# Autodesk Inventor assembly: default_motor_asembly
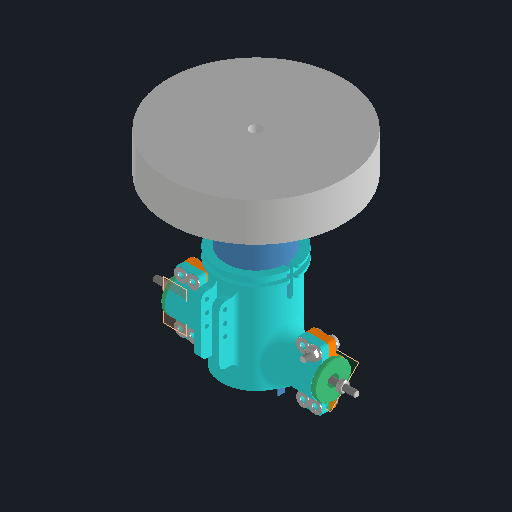
[picture p0: Inventor's stored thumbnail of the model, 512x512]
Saved by Autodesk Inventor 2024 (Build 280153000, 153)
## iProperties
Created: 2023-05-13
Part Number: default_motor_asembly
Document SubType Name: Assembly
Designer: user
Author: user
## Documents named in this file (9)
- D:\Docs\Robot\3d\motor_assembly\default_motor_asembly.iam
- D:\Docs\Robot\3d\motor_assembly\default_motor_asembly\lower_arm.ipt
- D:\Docs\Robot\3d\motor_assembly\default_motor_asembly\cup.ipt
- D:\Docs\Robot\3d\motor_assembly\bushing_assembly.iam
- D:\Docs\Robot\3d\default_components\motor.ipt
- C:\Users\user\Documents\Inventor\Content Center Files\R2024\ru-RU\DIN 125-1  A\DIN 125 - A 4,3.ipt
- C:\Users\user\Documents\Inventor\Content Center Files\R2024\ru-RU\DIN 7985 (H)\DIN 7985 (H) - M4x20-H.ipt
- C:\Users\user\Documents\Inventor\Content Center Files\R2024\ru-RU\DIN 934\DIN 934 - M4 x 0,7.ipt
- D:\Docs\Robot\3d\default_components\wheel.ipt
## Components (25 placed, 8 different names)
1. lower_arm:1 — Совмещение:1, Совмещение:2, Совмещение:3, Заподлицо:1, Вставка:2, Вставка:3, Вставка:4, Вставка:5, Вставка:6, Совмещение:4, Вставка:7, Вставка:8, Вставка:13, Вставка:14, Вставка:15, Вставка:16
2. cup:1 — Заподлицо:1, Вставка:1, Вставка:9, Вставка:10, Вставка:11, Вставка:12
3. bushing_assembly:1 [sub-assembly] — Вставка:1
4. bushing_assembly:2 [sub-assembly] — Вставка:2
5. cup:2 — Вставка:3, Вставка:4, Вставка:17, Вставка:18, Вставка:19, Вставка:20
6. motor:1 — Вставка:5, Вставка:23
7. DIN 125-1 A A 4,3:1 — Вставка:6
8. DIN 125-1 A A 4,3:2 — Совмещение:4
9. DIN 125-1 A A 4,3:3 — Вставка:8
10. DIN 125-1 A A 4,3:4 — Вставка:7
11. DIN 125-1 A A 4,3:5 — Вставка:9
12. DIN 125-1 A A 4,3:6 — Вставка:11
13. DIN 125-1 A A 4,3:7 — Вставка:12
14. DIN 125-1 A A 4,3:8 — Вставка:10
15. DIN 125-1 A A 4,3:9 — Вставка:13, Вставка:22
16. DIN 125-1 A A 4,3:10 — Вставка:14
17. DIN 125-1 A A 4,3:11 — Вставка:15
18. DIN 125-1 A A 4,3:12 — Вставка:16
19. DIN 125-1 A A 4,3:13 — Вставка:17
20. DIN 125-1 A A 4,3:14 — Вставка:18
21. DIN 125-1 A A 4,3:15 — Вставка:19
22. DIN 125-1 A A 4,3:16 — Вставка:20, Вставка:21
23. DIN 7985 (H) M4x20-H:1 — Вставка:21
24. DIN 934 - заменено на DIN EN 24032/28673/28674 M4:1 — Вставка:22
25. wheel:1 — Вставка:23
## Relationships (28: Insert 23, Mate 4, Flush 1)
- Совмещение:1 [Mate]: lower_arm:1
- Совмещение:2 [Mate]: lower_arm:1
- Совмещение:3 [Mate]: lower_arm:1
- Заподлицо:1 [Flush]: lower_arm:1 ↔ cup:1
- Вставка:1 [Insert]: cup:1 ↔ bushing_assembly:1
- Вставка:2 [Insert]: lower_arm:1 ↔ bushing_assembly:2
- Вставка:3 [Insert]: lower_arm:1 ↔ cup:2
- Вставка:4 [Insert]: lower_arm:1 ↔ cup:2
- Вставка:5 [Insert]: lower_arm:1 ↔ motor:1
- Вставка:6 [Insert]: lower_arm:1 ↔ DIN 125-1 A A 4,3:1
- Совмещение:4 [Mate]: lower_arm:1 ↔ DIN 125-1 A A 4,3:2
- Вставка:7 [Insert]: lower_arm:1 ↔ DIN 125-1 A A 4,3:4
- Вставка:8 [Insert]: lower_arm:1 ↔ DIN 125-1 A A 4,3:3
- Вставка:9 [Insert]: cup:1 ↔ DIN 125-1 A A 4,3:5
- Вставка:10 [Insert]: cup:1 ↔ DIN 125-1 A A 4,3:8
- Вставка:11 [Insert]: cup:1 ↔ DIN 125-1 A A 4,3:6
- Вставка:12 [Insert]: cup:1 ↔ DIN 125-1 A A 4,3:7
- Вставка:13 [Insert]: lower_arm:1 ↔ DIN 125-1 A A 4,3:9
- Вставка:14 [Insert]: lower_arm:1 ↔ DIN 125-1 A A 4,3:10
- Вставка:15 [Insert]: lower_arm:1 ↔ DIN 125-1 A A 4,3:11
- Вставка:16 [Insert]: lower_arm:1 ↔ DIN 125-1 A A 4,3:12
- Вставка:17 [Insert]: cup:2 ↔ DIN 125-1 A A 4,3:13
- Вставка:18 [Insert]: cup:2 ↔ DIN 125-1 A A 4,3:14
- Вставка:19 [Insert]: cup:2 ↔ DIN 125-1 A A 4,3:15
- Вставка:20 [Insert]: cup:2 ↔ DIN 125-1 A A 4,3:16
- Вставка:21 [Insert]: DIN 125-1 A A 4,3:16 ↔ DIN 7985 (H) M4x20-H:1
- Вставка:22 [Insert]: DIN 125-1 A A 4,3:9 ↔ DIN 934 - заменено на DIN EN 24032/28673/28674 M4:1
- Вставка:23 [Insert]: motor:1 ↔ wheel:1
